# Autodesk Inventor assembly: Ensamble
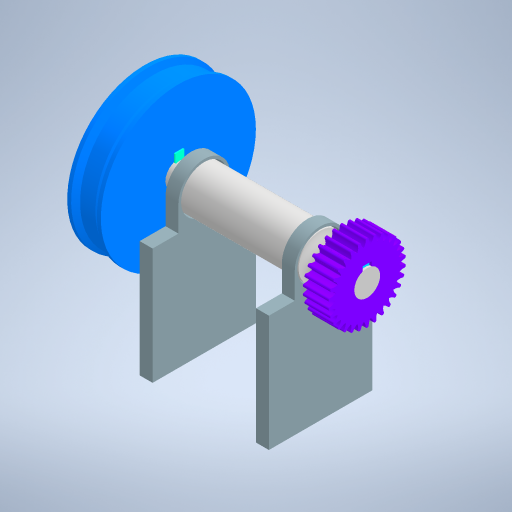
[picture p0: Inventor's stored thumbnail of the model, 512x512]
Saved by Autodesk Inventor 2024 (Build 280153000, 153)
## iProperties
Created: 2024-03-07
Part Number: Ensamble
Document SubType Name: Assembly
Designer: 50254
Author: 50254
## Documents named in this file (6)
- C:\Users\50254\Documents\Varios Daniela\Ingeniería Industrial\2024\Dinámica\Ensamble.iam
- C:\Users\50254\Downloads\POLEA.ipt
- C:\Users\50254\Downloads\ENGRANE.ipt
- C:\Users\50254\Downloads\EJE_CUÑEROS.ipt
- C:\Users\50254\Downloads\CUÑA.ipt
- C:\Users\50254\Documents\Varios Daniela\Ingeniería Industrial\2024\Dinámica\Soporte ensamble.ipt
## Components (7 placed, 5 different names)
1. POLEA:1 — Rígido:1
2. ENGRANE:1 — De rotación:1
3. EJE_CUÑEROS:1 — Rígido:1, De rotación:1, Rígido:2, Rígido:3, De rotación:2, Rígido:4
4. CUÑA:1 — Rígido:2
5. CUÑA:2 — Rígido:3
6. Soporte ensamble:1 — De rotación:2
7. Soporte ensamble:2 — Rígido:4
## Relationships (6: WeldJoint 4, RevoluteJoint 2)
- Rígido:1 [WeldJoint]: POLEA:1 ↔ EJE_CUÑEROS:1
- De rotación:1 [RevoluteJoint]: ENGRANE:1 ↔ EJE_CUÑEROS:1
- Rígido:2 [WeldJoint]: EJE_CUÑEROS:1 ↔ CUÑA:1
- Rígido:3 [WeldJoint]: EJE_CUÑEROS:1 ↔ CUÑA:2
- De rotación:2 [RevoluteJoint]: EJE_CUÑEROS:1 ↔ Soporte ensamble:1
- Rígido:4 [WeldJoint]: EJE_CUÑEROS:1 ↔ Soporte ensamble:2
